# Autodesk Inventor assembly: Shape Strip Test
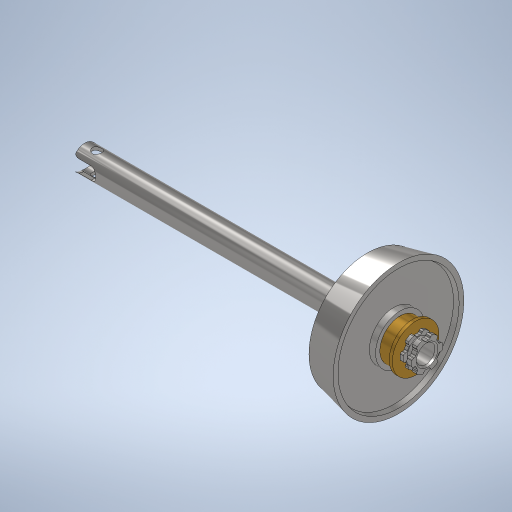
[picture p0: Inventor's stored thumbnail of the model, 512x512]
Saved by Autodesk Inventor 2023.2 (Build 272271000, 271)
## iProperties
Created: 2024-01-31
Part Number: Shape Strip Test
Document SubType Name: Assembly
Designer: Nathan Cai
Author: Nathan Cai
## Documents named in this file (10)
- E:\Documents\Inventor\Misc\Shape Strip Test.iam
- E:\Documents\Inventor\Misc\Bushing.ipt
- E:\Documents\Inventor\Misc\Shaft.ipt
- E:\Documents\Inventor\Misc\Clutch.ipt
- E:\Documents\Inventor\Misc\Shape Strip Test\AIP\FEA\elf48ahs0.fins
- E:\Documents\Inventor\Misc\Shape Strip Test\AIP\FEA\elf48ahs0.fsat
- E:\Documents\Inventor\Misc\Shape Strip Test\AIP\FEA\elf48ahs0.ftes
- E:\Documents\Inventor\Misc\Shape Strip Test\AIP\FEA\elf48ahs0.fwiz
- E:\Documents\Inventor\Misc\Shape Strip Test\AIP\FEA\elf48ahuo.fmsh
- E:\Documents\Inventor\Misc\Shape Strip Test\AIP\FEA\elf48ahup.fres
## Components (3 placed, 3 different names)
1. Bushing:1 — Mate:1, Flush:1, Mate:4, Mate:5, Mate:6
2. Shaft:1 — Mate:1, Flush:1, Mate:3, Mate:6
3. Clutch:1 — Mate:3, Mate:4, Mate:5
## Relationships (6: Mate 5, Flush 1)
- Mate:1: Bushing:1 ↔ Shaft:1
- Flush:1 (1 mm): Bushing:1 ↔ Shaft:1
- Mate:3: Shaft:1 ↔ Clutch:1
- Mate:4: Bushing:1 ↔ Clutch:1
- Mate:5: Bushing:1 ↔ Clutch:1
- Mate:6: Bushing:1 ↔ Shaft:1
## Named parameters: sa_0 = 225970
note: some values were not read from the file. Shown as the stored number, unit unknown: "sa_0".
